# Autodesk Inventor assembly: whole_assembly
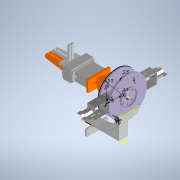
[picture p0: Inventor's stored thumbnail of the model, 180x180]
Saved by Autodesk Inventor 2021 (Build 250183000, 183)
## iProperties
Created: 2023-03-20
Part Number: whole_assembly
Document SubType Name: Assembly
Designer: mahmo
Author: mahmo
## Documents named in this file (10)
- D:\AsU\semesters\senior 2\new_gripper\whole_assembly.iam
- D:\AsU\semesters\senior 2\new_gripper\3dfindit-Festo-539636_HGP-16-A-B-SSK---_asm_0_-ZH_-0202303061711339323165410e898ce\AIS2021\539636 HGP-16-A-B-SSK---(asm_0_-ZH).iam
- D:\AsU\semesters\senior 2\new_gripper\tool_holder.ipt
- D:\AsU\semesters\senior 2\new_gripper\Part3.ipt
- D:\AsU\semesters\senior 2\new_gripper\suction_cup_holder.ipt
- D:\AsU\semesters\senior 2\new_gripper\manga.ipt
- D:\AsU\semesters\senior 2\new_gripper\normal_finger.ipt
- D:\AsU\semesters\senior 2\new_gripper\reverse_finger.ipt
- D:\AsU\semesters\senior 2\new_gripper\d435 i\Intel Realsense D435.ipt
- D:\AsU\semesters\senior 2\new_gripper\suction_cup_holder_MIR.ipt
## Components (11 placed, 9 different names)
1. 539636 HGP-16-A-B-SSK---(asm_0_-ZH):1 [sub-assembly] — Mate:1, Mate:2, Mate:7, Flush:4, Mate:23, Mate:24, Flush:8, Flush:9, Mate:37, Mate:38, Mate:39, Mate:40, Mate:47, Mate:59, Mate:62, Mate:63
2. tool_holder:1 — Mate:1, Mate:2, Mate:3, Mate:6, Flush:1, Mate:20, Mate:21, Mate:35, Mate:36
3. Part3:1 — Mate:3, Mate:6, Flush:1, Mate:7, Mate:34, Flush:10, Mate:45
4. manga:1 — Mate:20, Mate:21, Angle:1
5. normal_finger:1 — Flush:4, Mate:23, Mate:24, Mate:41
6. suction_cup_holder:2 — Mate:34, Mate:35, Mate:43, Mate:44
7. reverse_finger:1 — Mate:39, Mate:40, Mate:41, Mate:64
8. reverse_finger:2 — Mate:37, Mate:38
9. Intel Realsense D435:1 — Angle:1
10. normal_finger:2 — Mate:63, Mate:64
11. suction_cup_holder_MIR:1 — Mate:65, Mate:66
## Relationships (38: Mate 32, Flush 5, Angle 1)
- Mate:1: 539636 HGP-16-A-B-SSK---(asm_0_-ZH):1 ↔ tool_holder:1
- Mate:2: 539636 HGP-16-A-B-SSK---(asm_0_-ZH):1 ↔ tool_holder:1
- Mate:3: tool_holder:1 ↔ Part3:1
- Mate:6: tool_holder:1 ↔ Part3:1
- Flush:1: tool_holder:1 ↔ Part3:1
- Mate:7: 539636 HGP-16-A-B-SSK---(asm_0_-ZH):1 ↔ Part3:1
- Mate:20: tool_holder:1 ↔ manga:1
- Mate:21: tool_holder:1 ↔ manga:1
- Flush:4: 539636 HGP-16-A-B-SSK---(asm_0_-ZH):1 ↔ normal_finger:1
- Mate:23: 539636 HGP-16-A-B-SSK---(asm_0_-ZH):1 ↔ normal_finger:1
- Mate:24: 539636 HGP-16-A-B-SSK---(asm_0_-ZH):1 ↔ normal_finger:1
- Mate:34: Part3:1 ↔ suction_cup_holder:2
- Mate:35: tool_holder:1 ↔ suction_cup_holder:2
- Mate:36: tool_holder:1
- Flush:8: 539636 HGP-16-A-B-SSK---(asm_0_-ZH):1
- Flush:9: 539636 HGP-16-A-B-SSK---(asm_0_-ZH):1
- Flush:10: Part3:1
- Mate:37: 539636 HGP-16-A-B-SSK---(asm_0_-ZH):1 ↔ reverse_finger:2
- Mate:38: 539636 HGP-16-A-B-SSK---(asm_0_-ZH):1 ↔ reverse_finger:2
- Mate:39: 539636 HGP-16-A-B-SSK---(asm_0_-ZH):1 ↔ reverse_finger:1
- Mate:40: 539636 HGP-16-A-B-SSK---(asm_0_-ZH):1 ↔ reverse_finger:1
- Mate:41: normal_finger:1 ↔ reverse_finger:1
- Mate:43: suction_cup_holder:2
- Mate:44: suction_cup_holder:2
- Mate:45: Part3:1
- Mate:46
- Mate:47: 539636 HGP-16-A-B-SSK---(asm_0_-ZH):1
- Mate:53
- Mate:57
- Mate:58
- Mate:59: 539636 HGP-16-A-B-SSK---(asm_0_-ZH):1
- Mate:60
- Mate:62: 539636 HGP-16-A-B-SSK---(asm_0_-ZH):1
- Angle:1 (0 deg): manga:1 ↔ Intel Realsense D435:1
- Mate:63: 539636 HGP-16-A-B-SSK---(asm_0_-ZH):1 ↔ normal_finger:2
- Mate:64: reverse_finger:1 ↔ normal_finger:2
- Mate:65: suction_cup_holder_MIR:1
- Mate:66: suction_cup_holder_MIR:1
